# Autodesk Inventor assembly: FloorRoller
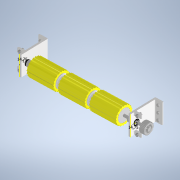
[picture p0: Inventor's stored thumbnail of the model, 180x180]
Saved by Autodesk Inventor 2021 (Build 250183000, 183)
## iProperties
Created: 2021-05-21
Part Number: FloorRoller
Document SubType Name: Assembly
Designer: sami8
Author: sami8
## Documents named in this file (12)
- C:\Users\sami8\Documents\SGD-FTC2021\CAD\FloorRoller\FloorRoller.iam
- C:\Users\sami8\Documents\SGD-FTC2021\CAD\FloorRoller\FlexRoller.ipt
- C:\Users\sami8\Documents\SGD-FTC2021\CAD\SolidRoller.ipt
- C:\Users\sami8\Documents\SGD-FTC2021\CAD\FloorRoller\MainHexShaft.ipt
- C:\Users\sami8\Documents\SGD-FTC2021\CAD\FloorRoller\REV-41-1326.ipt
- C:\Users\sami8\Documents\SGD-FTC2021\CAD\FloorRoller\REV-49-1559.ipt
- C:\Users\sami8\Documents\SGD-FTC2021\CAD\FloorRoller\REV-41-1123.ipt
- C:\Users\sami8\Documents\SGD-FTC2021\CAD\Base\REV-41-1361 Simple.ipt
- C:\Users\sami8\Documents\SGD-FTC2021\CAD\FloorRoller\BearingBracket.ipt
- C:\Users\sami8\Documents\SGD-FTC2021\CAD\SolidRollerNoPulley.ipt
- C:\Users\sami8\Documents\SGD-FTC2021\CAD\Base\REV-41-1327.ipt
- C:\Users\sami8\Documents\SGD-FTC2021\CAD\FloorRoller\REV-41-1332.ipt
## Components (36 placed, 11 different names)
1. BearingBracket:2 — Rigid:13, Rigid:14, Rigid:15, Rigid:16, Rigid:17, Rigid:18, Rigid:19, Rigid:20, Rigid:21, Rigid:22, Flush:1, Rigid:45, Rigid:46, Angle:1, Rigid:56
2. BearingBracket:3 — Rotational:1, Flush:1, Rigid:27, Rigid:28, Rigid:29, Rigid:30, Rigid:31, Rigid:32, Rigid:33, Rigid:34, Rigid:35, Rigid:36, Rigid:45
3. MainHexShaft:1 — Mate:4, Mate:5, Rigid:53, Angle:1
4. REV-41-1326:1 — Rigid:11, Rigid:43, Rigid:53
5. REV-49-1559:1 — Rigid:11, Rotational:1
6. REV-41-1327:1 — Rigid:43
7. REV-49-1559:2 — Rigid:46
8. REV-41-1326:2 — Rigid:55
9. REV-41-1327:2 — Rigid:55
10. REV-41-1332:1 — Rigid:56
11. REV-41-1361 Simple:10 — Rigid:34
12. REV-41-1361 Simple:9 — Rigid:36
13. REV-41-1361 Simple:8 — Rigid:30
14. REV-41-1361 Simple:7 — Rigid:28
15. REV-41-1361 Simple:6 — Rigid:32
16. REV-41-1123:13 — Rigid:31
17. REV-41-1123:12 — Rigid:29
18. REV-41-1123:11 — Rigid:33
19. REV-41-1123:10 — Rigid:35
20. REV-41-1123:9 — Rigid:27
21. REV-41-1123:1 — Rigid:20
22. REV-41-1123:2 — Rigid:19
23. REV-41-1123:3 — Rigid:18
24. REV-41-1123:4 — Rigid:21
25. REV-41-1123:5 — Rigid:22
26. REV-41-1361 Simple:1 — Rigid:13
27. REV-41-1361 Simple:2 — Rigid:17
28. REV-41-1361 Simple:3 — Rigid:15
29. REV-41-1361 Simple:4 — Rigid:14
30. REV-41-1361 Simple:5 — Rigid:16
31. FlexRoller:1 — Rigid:7
32. FlexRoller:2 — Rigid:40
33. FlexRoller:3 — Rigid:4
34. SolidRoller:2 — Rigid:4, Rigid:38
35. SolidRollerNoPulley:1 — Rigid:38, Rigid:39, Rigid:40
36. SolidRoller:3 — Rigid:7, Rigid:39, Mate:4, Mate:5
## Relationships (38: WeldJoint 33, Mate 2, RevoluteJoint 1, Flush 1, Angle 1)
- Rigid:4 [WeldJoint] (0.25 mm): FlexRoller:3 ↔ SolidRoller:2
- Rigid:7 [WeldJoint] (0.25 mm): FlexRoller:1 ↔ SolidRoller:3
- Rigid:11 [WeldJoint]: REV-41-1326:1 ↔ REV-49-1559:1
- Rigid:13 [WeldJoint]: BearingBracket:2 ↔ REV-41-1361 Simple:1
- Rigid:14 [WeldJoint]: BearingBracket:2 ↔ REV-41-1361 Simple:4
- Rigid:15 [WeldJoint]: BearingBracket:2 ↔ REV-41-1361 Simple:3
- Rigid:16 [WeldJoint]: BearingBracket:2 ↔ REV-41-1361 Simple:5
- Rigid:17 [WeldJoint]: BearingBracket:2 ↔ REV-41-1361 Simple:2
- Rigid:18 [WeldJoint] (-1.2 mm): BearingBracket:2 ↔ REV-41-1123:3
- Rigid:19 [WeldJoint] (-1.2 mm): BearingBracket:2 ↔ REV-41-1123:2
- Rigid:20 [WeldJoint] (-1.2 mm): BearingBracket:2 ↔ REV-41-1123:1
- Rigid:21 [WeldJoint] (-1.2 mm): BearingBracket:2 ↔ REV-41-1123:4
- Rigid:22 [WeldJoint] (-1.2 mm): BearingBracket:2 ↔ REV-41-1123:5
- Rotational:1 [RevoluteJoint]: BearingBracket:3 ↔ REV-49-1559:1
- Flush:1: BearingBracket:2 ↔ BearingBracket:3
- Rigid:27 [WeldJoint] (-1.2 mm): BearingBracket:3 ↔ REV-41-1123:9
- Rigid:28 [WeldJoint]: BearingBracket:3 ↔ REV-41-1361 Simple:7
- Rigid:29 [WeldJoint] (-1.2 mm): BearingBracket:3 ↔ REV-41-1123:12
- Rigid:30 [WeldJoint]: BearingBracket:3 ↔ REV-41-1361 Simple:8
- Rigid:31 [WeldJoint] (-1.2 mm): BearingBracket:3 ↔ REV-41-1123:13
- Rigid:32 [WeldJoint]: BearingBracket:3 ↔ REV-41-1361 Simple:6
- Rigid:33 [WeldJoint] (-1.2 mm): BearingBracket:3 ↔ REV-41-1123:11
- Rigid:34 [WeldJoint]: BearingBracket:3 ↔ REV-41-1361 Simple:10
- Rigid:35 [WeldJoint] (-1.2 mm): BearingBracket:3 ↔ REV-41-1123:10
- Rigid:36 [WeldJoint]: BearingBracket:3 ↔ REV-41-1361 Simple:9
- Rigid:38 [WeldJoint]: SolidRoller:2 ↔ SolidRollerNoPulley:1
- Rigid:39 [WeldJoint]: SolidRollerNoPulley:1 ↔ SolidRoller:3
- Rigid:40 [WeldJoint] (0.25 mm): FlexRoller:2 ↔ SolidRollerNoPulley:1
- Rigid:43 [WeldJoint] (-0.237 mm): REV-41-1326:1 ↔ REV-41-1327:1
- [WeldJoint]: REV-49-1559:2 ↔ REV-41-1326:2
- Rigid:45 [WeldJoint] (240 mm): BearingBracket:2 ↔ BearingBracket:3
- Rigid:46 [WeldJoint]: BearingBracket:2 ↔ REV-49-1559:2
- Mate:4: MainHexShaft:1 ↔ SolidRoller:3
- Mate:5: MainHexShaft:1 ↔ SolidRoller:3
- Rigid:53 [WeldJoint]: MainHexShaft:1 ↔ REV-41-1326:1
- Rigid:55 [WeldJoint] (0.237 mm): REV-41-1326:2 ↔ REV-41-1327:2
- Angle:1 (0 deg): BearingBracket:2 ↔ MainHexShaft:1
- Rigid:56 [WeldJoint] (-15 mm): BearingBracket:2 ↔ REV-41-1332:1
## Named parameters: d57_d20 = 0 mm
